# Autodesk Inventor assembly: Shell
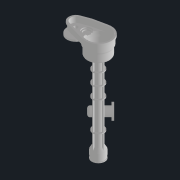
[picture p0: Inventor's stored thumbnail of the model, 180x180]
Saved by Autodesk Inventor 2021 (Build 250183000, 183)
## iProperties
Created: 2020-10-12
Part Number: Shell
Document SubType Name: Assembly
Designer: Eugene Tang
Mass: 1299.37 g
Surface Area: 4920.1 cm^2
Volume: 1299.37 cm^3
Density: 1 g/cm^3
Author: Eugene Tang
## Documents named in this file (7)
- C:\Users\teuge\OneDrive - Curtin University of Technology Australia\Y4S2\DFM\Group Project\CAD\Master\Shell.iam
- C:\Users\teuge\OneDrive - Curtin University of Technology Australia\Y4S2\DFM\Group Project\CAD\Master\Screw.ipt
- C:\Users\teuge\OneDrive - Curtin University of Technology Australia\Y4S2\DFM\Group Project\CAD\Master\Steering Gear.ipt
- C:\Users\teuge\OneDrive - Curtin University of Technology Australia\Y4S2\DFM\Group Project\CAD\Master\Shell.ipt
- C:\Users\teuge\OneDrive - Curtin University of Technology Australia\Y4S2\DFM\Group Project\CAD\Parts\Ball Screw Nut 1.0.ipt
- C:\Users\teuge\OneDrive - Curtin University of Technology Australia\Y4S2\DFM\Group Project\CAD\Master\Ball Screw Assembly\Design Accelerator\Spur Gear12.ipt
- E:\Y4S2\DFM\Group Project\Parameters.xlsx
## Components (1 placed, 1 different names)
1. Shell:1
## Named parameters: TD = 0.5, Ball_DIA = 6.35 mm, Screw_L = 292 mm, Screw_DIA = 36 mm, Screw_PITCH = 1 mm, Screw_LEAD = 10 mm, Nut_L = 80 mm, Nut_OD = 66 mm, Flange_OFFSET = 50 mm, Flange_DIA = 80 mm, Flange_L = 10 mm, BPath_REVQ = 5.75, Tread_OFFSET = 8.405 mm, TotalSteeringColumn_L = 840 mm, FSteeringColumn_L = 100 mm, RSteeringColumn_L = 80 mm, SteeringColumnChamfer_DEG = 20 deg, Rack_L = 307.252 mm, SteeringColumn_DIA = 26 mm, contact = 26 mm, rack_DEPTH = 6 mm, ToothH = 5.62 mm, SteererGearPlane = 18.76 mm, GearLength = 45 mm, NutCapTread_L = 25 mm, NutCapTread_THICKNESS = 5 mm, NutCap_OD = 60 mm, Gear_Thickness = 50 mm, GearToHub_Ratio = 0.6, GearThickness = 50 mm, GeartoHub_Ratio = 0.6, Facewidth = 30 mm, Tread_OD = 46 mm, Hub_L = 10 mm, SupportFlange_THICKNESS = 5 mm
